# Autodesk Inventor assembly: Untitled
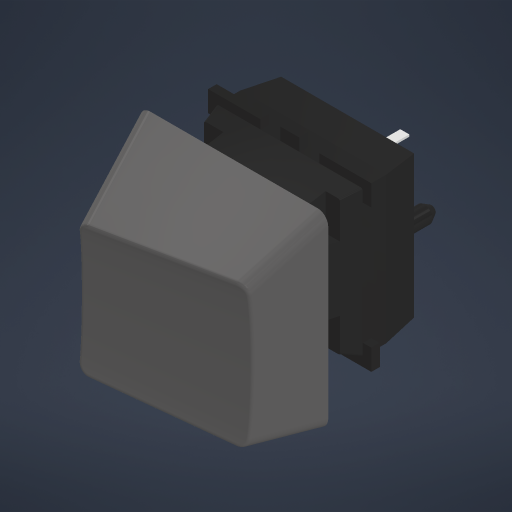
[picture p0: Inventor's stored thumbnail of the model, 512x512]
Saved by Autodesk Inventor 2024 (Build 280153000, 153)
## iProperties
Created: 2026-06-20
Part Number: Untitled
Document SubType Name: Assembly
Designer: schar
Sending System: Autodesk Translation Framework v15.8.0.0
Preprocessor: ST-DEVELOPER v20.1
Title: aneesh's stupid keycap for his master.step
## Documents named in this file (3)
- C:\Users\schar\Projects\Badge\foxbadge\cad\assets\key_asm.iam
- F:\aneesh's stupid keycap for his master\switch v1.iam
- F:\aneesh's stupid keycap for his master\Cherry MX keycaps v1.iam
## Components (2 placed, 2 different names)
1. switch v1:1 [sub-assembly] — Mate:1, Mate:2, Mate:3
2. Cherry MX keycaps v1:1 [sub-assembly] — Mate:1, Mate:2, Mate:3
## Relationships (3: Mate 3)
- Mate:1: switch v1:1 ↔ Cherry MX keycaps v1:1
- Mate:2: switch v1:1 ↔ Cherry MX keycaps v1:1
- Mate:3: switch v1:1 ↔ Cherry MX keycaps v1:1
